# Autodesk Inventor assembly: subsystem sorter finale
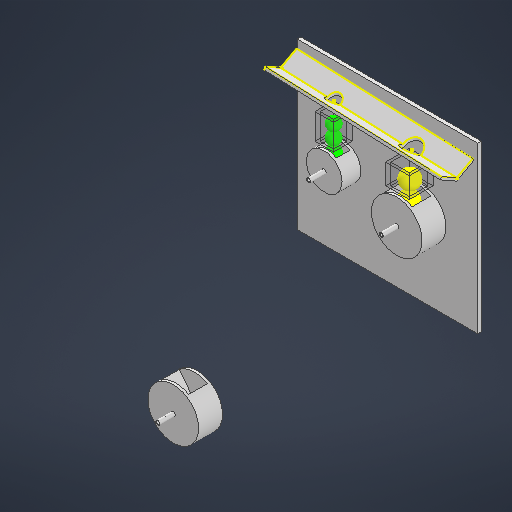
[picture p0: Inventor's stored thumbnail of the model, 512x512]
Saved by Autodesk Inventor 2026.1 (Build 301233020, 233B)
## iProperties
Created: 2026-05-04
Part Number: subsystem sorter finale
Document SubType Name: Assembly
Designer: hp
Author: hp
## Documents named in this file (10)
- C:\Users\hp\OneDrive\Documents\Inventor\BOM\subsystem sorter finale.iam
- C:\Users\hp\OneDrive\Documents\Inventor\BOM\sorternew.ipt
- C:\Users\hp\OneDrive\Documents\Inventor\BOM\new base for sorter.ipt
- C:\Users\hp\OneDrive\Documents\Inventor\BOM\ball holder small.ipt
- C:\Users\hp\OneDrive\Documents\Inventor\BOM\selector small.ipt
- C:\Users\hp\OneDrive\Documents\Inventor\BOM\green small ball.ipt
- C:\Users\hp\OneDrive\Documents\Inventor\BOM\servo motor.ipt
- C:\Users\hp\OneDrive\Documents\Inventor\BOM\ball holder medium.ipt
- C:\Users\hp\OneDrive\Documents\Inventor\BOM\medium yellow ball.ipt
- C:\Users\hp\OneDrive\Documents\Inventor\BOM\selector medium.ipt
## Components (14 placed, 9 different names)
1. sorternew:1 — Mate:1, Mate:2
2. new base for sorter:1 — Mate:1, Mate:2, Mate:3, Mate:4, Mate:5, Mate:6, Mate:7, Mate:8
3. ball holder small:1
4. green small ball:1
5. green small ball:2
6. green small ball:3
7. ball holder medium:1
8. medium yellow ball:2
9. servo motor:1 — Mate:3, Mate:4, Mate:5, Mate:9, Mate:10
10. servo motor:2 — Mate:6, Mate:7, Mate:8, Mate:11, Mate:12
11. selector small:1 — Mate:9, Mate:10
12. selector medium:1 — Mate:11, Mate:12
13. medium yellow ball:3
14. selector medium:2
## Relationships (12: Mate 12)
- Mate:1: sorternew:1 ↔ new base for sorter:1
- Mate:2: sorternew:1 ↔ new base for sorter:1
- Mate:3: new base for sorter:1 ↔ servo motor:1
- Mate:4: new base for sorter:1 ↔ servo motor:1
- Mate:5: new base for sorter:1 ↔ servo motor:1
- Mate:6: new base for sorter:1 ↔ servo motor:2
- Mate:7: new base for sorter:1 ↔ servo motor:2
- Mate:8: new base for sorter:1 ↔ servo motor:2
- Mate:9: servo motor:1 ↔ selector small:1
- Mate:10: servo motor:1 ↔ selector small:1
- Mate:11: servo motor:2 ↔ selector medium:1
- Mate:12: servo motor:2 ↔ selector medium:1
